# Autodesk Inventor assembly: Prototipo2
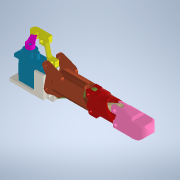
[picture p0: Inventor's stored thumbnail of the model, 180x180]
Saved by Autodesk Inventor 2020.4 (Build 244396010, 396A)
## iProperties
Created: 2021-08-13
Part Number: Prototipo2
Document SubType Name: Assembly
Designer: chalo
Author: chalo
## Documents named in this file (10)
- C:\Users\chalo\OneDrive\Documents\GitHub\Interfaces-Biomedicas-2021\Gonzalo Palarea\Inventor\tipo2\Prototipo2.iam
- C:\Users\chalo\OneDrive\Documents\GitHub\Interfaces-Biomedicas-2021\Gonzalo Palarea\Inventor\stls\Base_v2.ipt
- C:\Users\chalo\OneDrive\Documents\GitHub\Interfaces-Biomedicas-2021\Gonzalo Palarea\Inventor\servoconbrazo.iam
- C:\Users\chalo\OneDrive\Documents\GitHub\Interfaces-Biomedicas-2021\Gonzalo Palarea\Inventor\tipo2\Metacarpo.ipt
- C:\Users\chalo\OneDrive\Documents\GitHub\Interfaces-Biomedicas-2021\Gonzalo Palarea\Inventor\tipo2\Palanca servo_dedo_1.ipt
- C:\Users\chalo\OneDrive\Documents\GitHub\Interfaces-Biomedicas-2021\Gonzalo Palarea\Inventor\tipo2\Palanca servo_dedo_2.ipt
- C:\Users\chalo\OneDrive\Documents\GitHub\Interfaces-Biomedicas-2021\Gonzalo Palarea\Inventor\tipo2\Falange proxima.ipt
- C:\Users\chalo\OneDrive\Documents\GitHub\Interfaces-Biomedicas-2021\Gonzalo Palarea\Inventor\tipo2\palanca base_proxima.ipt
- C:\Users\chalo\OneDrive\Documents\GitHub\Interfaces-Biomedicas-2021\Gonzalo Palarea\Inventor\tipo2\Falange_media_distal.ipt
- C:\Users\chalo\OneDrive\Documents\GitHub\Interfaces-Biomedicas-2021\Gonzalo Palarea\Inventor\tipo2\Palanca metacarpo_distal.ipt
## Components (9 placed, 9 different names)
1. Base_v2:1 — Mate:1, Angle:1, Insert:1, Flush:1, Flush:2, Flush:7
2. servoconbrazo:1 [sub-assembly] — Mate:1, Angle:1, Insert:1, Flush:3, Flush:4, Flush:10
3. Metacarpo:1 — Flush:1, Flush:2, Flush:6, Flush:7, Flush:8
4. Palanca servo_dedo_1:1 — Flush:3, Flush:4, Flush:5
5. Palanca servo_dedo_2:1 — Flush:5
6. Falange proxima:1 — Flush:6, Flush:9
7. palanca base_proxima:1 — Flush:8
8. Falange_media_distal:1 — Flush:9
9. Palanca metacarpo_distal:1 — Flush:10
## Relationships (13: Flush 10, Mate 1, Angle 1, Insert 1)
- Mate:1: Base_v2:1 ↔ servoconbrazo:1
- Angle:1 (0 deg): Base_v2:1 ↔ servoconbrazo:1
- Insert:1: Base_v2:1 ↔ servoconbrazo:1
- Flush:1: Base_v2:1 ↔ Metacarpo:1
- Flush:2: Base_v2:1 ↔ Metacarpo:1
- Flush:3: servoconbrazo:1 ↔ Palanca servo_dedo_1:1
- Flush:4: servoconbrazo:1 ↔ Palanca servo_dedo_1:1
- Flush:5: Palanca servo_dedo_1:1 ↔ Palanca servo_dedo_2:1
- Flush:6: Metacarpo:1 ↔ Falange proxima:1
- Flush:7: Base_v2:1 ↔ Metacarpo:1
- Flush:8: Metacarpo:1 ↔ palanca base_proxima:1
- Flush:9: Falange proxima:1 ↔ Falange_media_distal:1
- Flush:10: servoconbrazo:1 ↔ Palanca metacarpo_distal:1
